# Autodesk Inventor assembly: Assembly4
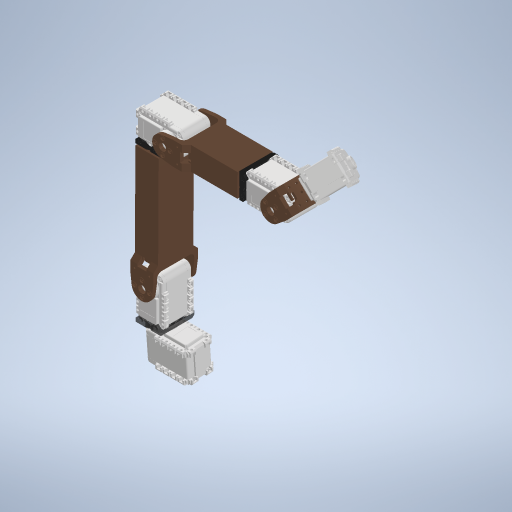
[picture p0: Inventor's stored thumbnail of the model, 512x512]
Saved by Autodesk Inventor 2024 (Build 280153000, 153)
## iProperties
Created: 2023-11-24
Part Number: Assembly4
Document SubType Name: Assembly
Designer: Anita
Author: Anita
## Documents named in this file (7)
- C:\Users\Anita\Desktop\Assembly4.iam
- C:\Users\Anita\Downloads\AX-12A\AX-12A.ipt
- C:\Users\Anita\Downloads\FP04-F2\FP04-F2.ipt
- C:\Users\Anita\Downloads\FP04-F3\FP04-F3.ipt
- C:\Users\Anita\Downloads\FP04-F3 (2)\FP04-F3 (2).ipt
- C:\Users\Anita\Downloads\FP04-F2_1.ipt
- C:\Users\Anita\Downloads\FP04-F2_3.ipt
## Components (11 placed, 6 different names)
1. AX-12A:1 — Symmetry:1, Mate:1, Mate:2, Mate:3, Mate:4, Mate:5
2. FP04-F2:1 — Symmetry:1, Mate:1, Mate:6, Mate:7, Mate:8
3. FP04-F3:1 — Mate:2, Mate:3, Mate:4, Mate:5, Mate:18, Mate:19
4. FP04-F3 (2):1 — Mate:6, Mate:7, Mate:8, Mate:9, Mate:10, Mate:11
5. AX-12A:2 — Mate:9, Mate:10, Mate:11, Rotational:1
6. AX-12A:3 — Mate:21, Mate:22
7. AX-12A:4 — Mate:15, Mate:16, Mate:17, Rotational:2, Mate:20
8. FP04-F2_1:1 — Rotational:1, Mate:12, Mate:13, Mate:14
9. FP04-F3:2 — Mate:12, Mate:13, Mate:14, Mate:15, Mate:16, Mate:17
10. AX-12A:5 — Mate:18, Mate:19
11. FP04-F2_3:1 — Rotational:2, Mate:20, Mate:21, Mate:22
## Relationships (25: Mate 22, RevoluteJoint 2, Symmetry 1)
- Symmetry:1: AX-12A:1 ↔ FP04-F2:1
- Mate:1: AX-12A:1 ↔ FP04-F2:1
- Mate:2: AX-12A:1 ↔ FP04-F3:1
- Mate:3: AX-12A:1 ↔ FP04-F3:1
- Mate:4: AX-12A:1 ↔ FP04-F3:1
- Mate:5: AX-12A:1 ↔ FP04-F3:1
- Mate:6: FP04-F2:1 ↔ FP04-F3 (2):1
- Mate:7: FP04-F2:1 ↔ FP04-F3 (2):1
- Mate:8: FP04-F2:1 ↔ FP04-F3 (2):1
- Mate:9: FP04-F3 (2):1 ↔ AX-12A:2
- Mate:10: FP04-F3 (2):1 ↔ AX-12A:2
- Mate:11: FP04-F3 (2):1 ↔ AX-12A:2
- Rotational:1 [RevoluteJoint]: AX-12A:2 ↔ FP04-F2_1:1
- Mate:12: FP04-F2_1:1 ↔ FP04-F3:2
- Mate:13: FP04-F2_1:1 ↔ FP04-F3:2
- Mate:14: FP04-F2_1:1 ↔ FP04-F3:2
- Mate:15: AX-12A:4 ↔ FP04-F3:2
- Mate:16: AX-12A:4 ↔ FP04-F3:2
- Mate:17: AX-12A:4 ↔ FP04-F3:2
- Mate:18: FP04-F3:1 ↔ AX-12A:5
- Mate:19: FP04-F3:1 ↔ AX-12A:5
- Rotational:2 [RevoluteJoint]: AX-12A:4 ↔ FP04-F2_3:1
- Mate:20: AX-12A:4 ↔ FP04-F2_3:1
- Mate:21: AX-12A:3 ↔ FP04-F2_3:1
- Mate:22: AX-12A:3 ↔ FP04-F2_3:1
